# Autodesk Inventor assembly: Rail_wheel_assembly
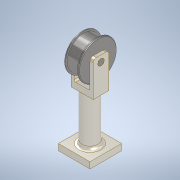
[picture p0: Inventor's stored thumbnail of the model, 180x180]
Saved by Autodesk Inventor 2022 (Build 260153000, 153)
## iProperties
Created: 2021-11-07
Part Number: Rail_wheel_assembly
Document SubType Name: Assembly
Designer: kibandi
Author: kibandi
## Documents named in this file (10)
- C:\academics\YEAR 4\4.2\DOMS II\DOMS II projects\mechanical design\Rail_wheel_assembly.iam
- C:\academics\YEAR 4\4.2\DOMS II\DOMS II projects\mechanical design\rail wheel.ipt
- C:\academics\YEAR 4\4.2\DOMS II\DOMS II projects\mechanical design\wheel connector.ipt
- C:\academics\YEAR 4\4.2\DOMS II\DOMS II projects\mechanical design\wheel_axle.ipt
- C:\academics\YEAR 4\4.2\DOMS II\DOMS II projects\mechanical design\Rail_wheel_assembly\AIP\FEA\ds7xbh1k0.fins
- C:\academics\YEAR 4\4.2\DOMS II\DOMS II projects\mechanical design\Rail_wheel_assembly\AIP\FEA\ds7xbh1kw.fsat
- C:\academics\YEAR 4\4.2\DOMS II\DOMS II projects\mechanical design\Rail_wheel_assembly\AIP\FEA\ds7xbh1kw.ftes
- C:\academics\YEAR 4\4.2\DOMS II\DOMS II projects\mechanical design\Rail_wheel_assembly\AIP\FEA\ds7xbh1kw.fwiz
- C:\academics\YEAR 4\4.2\DOMS II\DOMS II projects\mechanical design\Rail_wheel_assembly\AIP\FEA\ds7xbh1pc.fmsh
- C:\academics\YEAR 4\4.2\DOMS II\DOMS II projects\mechanical design\Rail_wheel_assembly\AIP\FEA\ds7xbh1q8.fres
## Components (3 placed, 3 different names)
1. rail wheel:1 — Mate:1, Mate:3
2. wheel connector:1 — Mate:2, Mate:3
3. wheel_axle:1 — Mate:1, Mate:2
## Relationships (3: Mate 3)
- Mate:1: rail wheel:1 ↔ wheel_axle:1
- Mate:2: wheel connector:1 ↔ wheel_axle:1
- Mate:3: rail wheel:1 ↔ wheel connector:1
## Named parameters: sa_0 = 70000
note: some values were not read from the file. Shown as the stored number, unit unknown: "sa_0".
